# Autodesk Inventor assembly: mesh-window-35mm-assembly
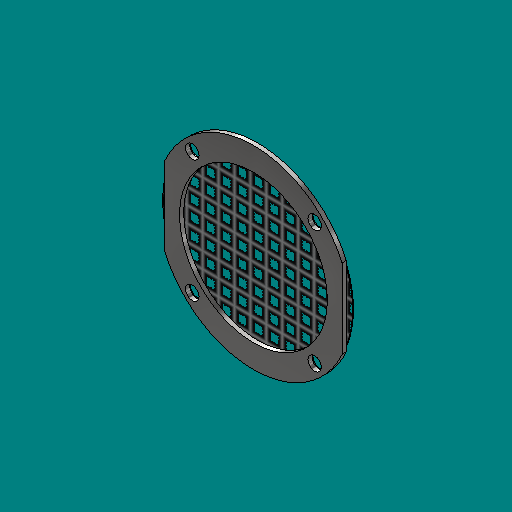
[picture p0: Inventor's stored thumbnail of the model, 512x512]
Saved by Autodesk Inventor 2025 (Build 290162000, 162)
## iProperties
Created: 2024-05-22
Part Number: mesh-window-35mm-assembly
Document SubType Name: Assembly
Designer: kuzmin
Mass: 7.11885 g
Surface Area: 45.7968 cm^2
Volume: 0.889856 cm^3
Density: 8 g/cm^3
Author: kuzmin
## Documents named in this file (5)
- C:\Users\queez\Dropbox\Drawings\PIHTI\Plasma Vessel\Plasma-Box\mesh-window-35mm-assembly.iam
- C:\Users\queez\Dropbox\Drawings\PIHTI\Plasma Vessel\Plasma-Box\probe-gate-spacer\probe-gate-spacer-straight-35mm.ipt
- C:\Users\queez\Dropbox\Drawings\PIHTI\Plasma Vessel\Plasma-Box\probe-gate-spacer.ipt
- C:\Users\queez\Dropbox\Drawings\PIHTI\Plasma Vessel\Plasma-Box\probe-gate-mesh-circle\probe-gate-mesh-circle-45mm.ipt
- C:\Users\queez\Dropbox\Drawings\PIHTI\Plasma Vessel\Plasma-Box\probe-gate-mesh-circle.ipt
## Components (2 placed, 2 different names)
1. probe-gate-spacer-straight-35mm:1 — Rotational:3, Mate:1
2. probe-gate-mesh-circle-45mm:1 — Rotational:3, Mate:1
## Relationships (2: RevoluteJoint 1, Mate 1)
- Rotational:3 [RevoluteJoint]: probe-gate-spacer-straight-35mm:1 ↔ probe-gate-mesh-circle-45mm:1
- Mate:1: probe-gate-spacer-straight-35mm:1 ↔ probe-gate-mesh-circle-45mm:1
